# Autodesk Inventor assembly: CameraCase
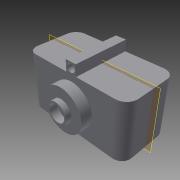
[picture p0: Inventor's stored thumbnail of the model, 180x180]
Saved by Autodesk Inventor 2015 SP1 (Build 190203100, 203)
## iProperties
Created: 2015-05-03
Part Number: CameraCase
Document SubType Name: Assembly
Designer: Brandon
Author: Brandon
## Documents named in this file (4)
- C:\Users\Brandon\Documents\GitHub\Edith\Case\Camera\CameraCase.iam
- C:\Users\Brandon\Documents\GitHub\Edith\Case\Camera\Back.ipt
- C:\Users\Brandon\Documents\GitHub\Edith\Case\Camera\Front.ipt
- C:\Users\Brandon\Documents\GitHub\Edith\Case\Camera\Lens.ipt
## Components (3 placed, 3 different names)
1. Back:1 — Flush:1, Flush:2
2. Front:1 — Flush:1, Flush:2, Flush:3
3. Lens:1 — Flush:3
## Relationships (3: Flush 3)
- Flush:1: Back:1 ↔ Front:1
- Flush:2: Back:1 ↔ Front:1
- Flush:3: Front:1 ↔ Lens:1
